# Autodesk Inventor assembly: carrier_board_2019-06-12
(part 2 of 2)
188. C39_382 [sub-assembly]
189. C40_384 [sub-assembly]
190. C79_386 [sub-assembly]
191. C81_388 [sub-assembly]
192. D39_390 [sub-assembly]
193. D40_392 [sub-assembly]
194. D41_394 [sub-assembly]
195. FU10_396 [sub-assembly]
196. FU9_398 [sub-assembly]
197. Q6_400 [sub-assembly]
198. R63_402 [sub-assembly]
199. R70_404 [sub-assembly]
200. R42_406 [sub-assembly]
201. R43_408 [sub-assembly]
202. R61_410 [sub-assembly]
203. R64_412 [sub-assembly]
204. C28_414 [sub-assembly]
205. C24_416 [sub-assembly]
206. C34_418 [sub-assembly]
207. C73_420 [sub-assembly]
208. D18_422 [sub-assembly]
209. D19_424 [sub-assembly]
210. D23_426 [sub-assembly]
211. U3_428 [sub-assembly]
212. U5_430 [sub-assembly]
213. R36_432 [sub-assembly]
214. R33_434 [sub-assembly]
215. FU6_436 [sub-assembly]
216. FU5_438 [sub-assembly]
217. D14_440 [sub-assembly]
218. D13_442 [sub-assembly]
219. D12_444 [sub-assembly]
220. C53_446 [sub-assembly]
221. C31_448 [sub-assembly]
222. C30_450 [sub-assembly]
223. C26_452 [sub-assembly]
224. C27_454 [sub-assembly]
225. R25_456 [sub-assembly]
226. R17_458 [sub-assembly]
227. C19_460 [sub-assembly]
228. C18_462 [sub-assembly]
229. C25_464 [sub-assembly]
230. C51_466 [sub-assembly]
231. D10_468 [sub-assembly]
232. D8_470 [sub-assembly]
233. FU3_472 [sub-assembly]
234. FU4_474 [sub-assembly]
235. Q3_476 [sub-assembly]
236. R21_478 [sub-assembly]
237. R30_480 [sub-assembly]
238. R16_482 [sub-assembly]
239. R20_484 [sub-assembly]
240. R24_486 [sub-assembly]
241. R160_488 [sub-assembly]
242. C100_490 [sub-assembly]
243. C102_492 [sub-assembly]
244. C110_494 [sub-assembly]
245. D27_496 [sub-assembly]
246. D28_498 [sub-assembly]
247. FB10_500 [sub-assembly]
248. FU19_502 [sub-assembly]
249. FU20_504 [sub-assembly]
250. R154_506 [sub-assembly]
251. R155_508 [sub-assembly]
252. R159_510 [sub-assembly]
253. R151_512 [sub-assembly]
254. R158_514 [sub-assembly]
255. R181_516 [sub-assembly]
256. D21_518 [sub-assembly]
257. R157_520 [sub-assembly]
258. R128_522 [sub-assembly]
259. R129_524 [sub-assembly]
260. R126_526 [sub-assembly]
261. R125_528 [sub-assembly]
262. R123_530 [sub-assembly]
263. FU14_532 [sub-assembly]
264. FU13_534 [sub-assembly]
265. FB4_536 [sub-assembly]
266. C104_538 [sub-assembly]
267. C86_540 [sub-assembly]
268. C84_542 [sub-assembly]
269. C88_544 [sub-assembly]
270. C90_546 [sub-assembly]
271. C103_548 [sub-assembly]
272. C108_550 [sub-assembly]
273. D20_552 [sub-assembly]
274. D22_554 [sub-assembly]
275. FB6_556 [sub-assembly]
276. FU15_558 [sub-assembly]
277. FU16_560 [sub-assembly]
278. R135_562 [sub-assembly]
279. R136_564 [sub-assembly]
280. R133_566 [sub-assembly]
281. R138_568 [sub-assembly]
282. R137_570 [sub-assembly]
283. R163_572 [sub-assembly]
284. CON2_574 [sub-assembly]
285. U11_576 [sub-assembly]
286. U10_578 [sub-assembly]
287. U7_580 [sub-assembly]
288. U20_582 [sub-assembly]
289. U19_584 [sub-assembly]
290. U18_586 [sub-assembly]
291. U17_588 [sub-assembly]
292. U1_590 [sub-assembly]
293. S1_592 [sub-assembly]
294. R6_594 [sub-assembly]
295. R162_596 [sub-assembly]
296. R152_598 [sub-assembly]
297. R164_600 [sub-assembly]
298. R147_602 [sub-assembly]
299. R149_604 [sub-assembly]
300. R143_606 [sub-assembly]
301. R140_608 [sub-assembly]
302. R134_610 [sub-assembly]
303. R120_612 [sub-assembly]
304. R130_614 [sub-assembly]
305. R124_616 [sub-assembly]
306. R122_618 [sub-assembly]
307. R121_620 [sub-assembly]
308. R142_622 [sub-assembly]
309. R146_624 [sub-assembly]
310. R145_626 [sub-assembly]
311. R87_628 [sub-assembly]
312. R84_630 [sub-assembly]
313. R83_632 [sub-assembly]
314. R76_634 [sub-assembly]
315. R112_636 [sub-assembly]
316. R113_638 [sub-assembly]
317. R73_640 [sub-assembly]
318. R103_642 [sub-assembly]
319. R102_644 [sub-assembly]
320. R101_646 [sub-assembly]
321. R62_648 [sub-assembly]
322. R97_650 [sub-assembly]
323. R60_652 [sub-assembly]
324. R59_654 [sub-assembly]
325. R91_656 [sub-assembly]
326. R90_658 [sub-assembly]
327. R77_660 [sub-assembly]
328. R72_662 [sub-assembly]
329. R53_664 [sub-assembly]
330. R52_666 [sub-assembly]
331. R86_668 [sub-assembly]
332. R78_670 [sub-assembly]
333. R75_672 [sub-assembly]
334. R44_674 [sub-assembly]
335. R40_676 [sub-assembly]
336. R35_678 [sub-assembly]
337. R14_680 [sub-assembly]
338. R7_682 [sub-assembly]
339. R18_684 [sub-assembly]
340. R11_686 [sub-assembly]
341. R1_688 [sub-assembly]
342. R5_690 [sub-assembly]
343. R4_692 [sub-assembly]
344. R3_694 [sub-assembly]
345. Q11_696 [sub-assembly]
346. Q10_698 [sub-assembly]
347. Q8_700 [sub-assembly]
348. Q7_702 [sub-assembly]
349. Q2_704 [sub-assembly]
350. Q1_706 [sub-assembly]
351. L3_708 [sub-assembly]
352. L2_710 [sub-assembly]
353. L1_712 [sub-assembly]
354. FU18_714 [sub-assembly]
355. FU17_716 [sub-assembly]
356. FU12_718 [sub-assembly]
357. FU11_720 [sub-assembly]
358. FU2_722 [sub-assembly]
359. FB8_724 [sub-assembly]
360. FB3_726 [sub-assembly]
361. FB2_728 [sub-assembly]
362. D50_730 [sub-assembly]
363. D49_732 [sub-assembly]
364. D47_734 [sub-assembly]
365. D45_736 [sub-assembly]
366. D44_738 [sub-assembly]
367. D30_740 [sub-assembly]
368. D29_742 [sub-assembly]
369. D25_744 [sub-assembly]
370. D16_746 [sub-assembly]
371. D2_748 [sub-assembly]
372. CON8_750 [sub-assembly]
373. CON6_752 [sub-assembly]
374. CON7_754 [sub-assembly]
375. CON5_756 [sub-assembly]
376. CON4_761 [sub-assembly]
377. CON3_763 [sub-assembly]
378. C82_765 [sub-assembly]
379. C38_767 [sub-assembly]
380. C106_769 [sub-assembly]
381. C105_771 [sub-assembly]
382. C107_773 [sub-assembly]
383. C99_775 [sub-assembly]
384. C98_777 [sub-assembly]
385. C109_779 [sub-assembly]
386. C93_781 [sub-assembly]
387. C92_783 [sub-assembly]
388. C83_785 [sub-assembly]
389. C95_787 [sub-assembly]
390. C49_789 [sub-assembly]
391. C89_791 [sub-assembly]
392. C87_793 [sub-assembly]
393. C44_795 [sub-assembly]
394. C43_797 [sub-assembly]
395. C96_799 [sub-assembly]
396. C94_801 [sub-assembly]
397. C68_803 [sub-assembly]
398. C67_805 [sub-assembly]
399. C66_807 [sub-assembly]
400. C65_809 [sub-assembly]
401. C62_811 [sub-assembly]
402. C61_813 [sub-assembly]
403. C60_815 [sub-assembly]
404. C59_817 [sub-assembly]
405. C57_819 [sub-assembly]
406. C56_821 [sub-assembly]
407. C69_823 [sub-assembly]
408. C54_825 [sub-assembly]
409. C52_827 [sub-assembly]
410. C50_829 [sub-assembly]
411. C41_831 [sub-assembly]
412. C17_833 [sub-assembly]
413. C16_835 [sub-assembly]
414. C14_837 [sub-assembly]
415. C15_839 [sub-assembly]
416. C13_841 [sub-assembly]
417. C12_843 [sub-assembly]
418. C11_845 [sub-assembly]
419. C10_847 [sub-assembly]
420. C9_849 [sub-assembly]
421. C8_851 [sub-assembly]
422. C7_853 [sub-assembly]
423. C6_855 [sub-assembly]
424. C5_857 [sub-assembly]
425. C4_859 [sub-assembly]
426. C3_861 [sub-assembly]
427. C1_863 [sub-assembly]
